# Autodesk Inventor assembly: 5-5
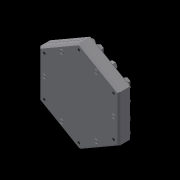
[picture p0: Inventor's stored thumbnail of the model, 180x180]
Saved by Autodesk Inventor 2017 (Build 210142000, 142)
## iProperties
Part Number: 5-5
Material: 一般
Document SubType Name: Assembly
Designer: r0909
Author: r0909
## Documents named in this file (7)
- C:\Users\r0909\Desktop\inventor\5-5.iam
- C:\Users\r0909\Desktop\inventor\5-1.ipt
- C:\Users\r0909\Desktop\inventor\5-2.ipt
- C:\Users\r0909\Desktop\inventor\5-3.ipt
- C:\Users\r0909\Desktop\inventor\5-4.ipt
- C:\Users\r0909\Desktop\inventor\5-5.1.ipt
- C:\Users\r0909\Desktop\inventor\5-5.2.ipt
## Components (44 placed, 6 different names)
1. 5-1:1 — 貼合:1, 貼合:2, 貼合:3, 貼合:30, 角度:19
2. 5-2:1 — 貼合:1, 貼合:2, 貼合:3, 貼合:4, 貼合:5, 貼合:6, 貼合:7, 貼合:8, 貼合:9, 齊平:1, 齊平:2, 齊平:3, 齊平:4, 齊平:5, 齊平:6, 貼合:12, 貼合:13, 角度:1, 貼合:24, 貼合:25, 貼合:26, 貼合:27, 貼合:28, 貼合:29, 角度:2, 貼合:31, 貼合:32, 貼合:33, 貼合:34, 貼合:35, 貼合:36, 貼合:37, 貼合:38, 貼合:39, 貼合:40, 貼合:41, 貼合:42, 貼合:43, 貼合:44, 貼合:45, 貼合:46, 貼合:47, 貼合:48, 貼合:49, 貼合:50, 貼合:51, 貼合:52, 貼合:53, 角度:6, 角度:11, 角度:12
3. 5-3:1 — 貼合:4, 齊平:1
4. 5-4:1 — 貼合:29, 貼合:30, 角度:2, 齊平:12, 齊平:13, 齊平:22, 角度:3
5. 5-3:2 — 貼合:5, 齊平:2
6. 5-3:3 — 貼合:6, 齊平:6
7. 5-3:4 — 貼合:7, 齊平:3
8. 5-3:5 — 貼合:8, 齊平:5
9. 5-3:6 — 貼合:9, 齊平:4
10. 5-5.1:1 — 貼合:10, 貼合:11, 貼合:13, 齊平:7
11. 5-5.2:1 — 貼合:10, 貼合:11, 貼合:12, 角度:1
12. 5-5.1:2 — 齊平:7, 齊平:8
13. 5-5.2:2 — 貼合:25
14. 5-5.1:3 — 齊平:8, 齊平:9
15. 5-5.2:3 — 貼合:24, 角度:7
16. 5-5.1:4 — 齊平:10, 齊平:11
17. 5-5.2:4 — 貼合:27
18. 5-5.1:5 — 齊平:9, 齊平:10
19. 5-5.2:5 — 貼合:26
20. 5-5.1:6 — 齊平:11
21. 5-5.2:6 — 貼合:28
22. 5-4:2 — 貼合:31, 齊平:22, 齊平:23, 角度:18
23. 5-4:3 — 貼合:34, 齊平:14, 角度:12, 角度:13
24. 5-4:4 — 貼合:33, 齊平:13, 齊平:14, 齊平:15, 齊平:16, 齊平:17, 角度:11
25. 5-4:5 — 貼合:32, 齊平:12, 角度:3, 角度:4
26. 5-4:6 — 貼合:35, 齊平:23, 齊平:24, 角度:17, 角度:18
27. 5-4:7 — 貼合:37, 齊平:24, 齊平:25, 角度:8, 角度:9
28. 5-4:8 — 貼合:36, 齊平:25, 齊平:26, 角度:6, 角度:7, 角度:8
29. 5-4:9 — 貼合:38, 齊平:16, 齊平:18
30. 5-4:10 — 貼合:39, 齊平:15
31. 5-4:11 — 貼合:48, 齊平:28, 齊平:29
32. 5-4:12 — 貼合:49, 齊平:32, 齊平:33, 角度:5
33. 5-4:13 — 貼合:47, 齊平:31, 角度:13, 角度:14, 角度:15
34. 5-4:14 — 貼合:46, 齊平:33, 齊平:34, 角度:4, 角度:5
35. 5-4:15 — 貼合:45, 齊平:34, 角度:16
36. 5-4:16 — 貼合:42, 齊平:20, 角度:10
37. 5-4:17 — 貼合:40, 齊平:17, 角度:22
38. 5-4:18 — 貼合:44, 齊平:21, 角度:15, 角度:16, 角度:17
39. 5-4:19 — 貼合:43, 齊平:19, 齊平:21, 角度:9, 角度:10
40. 5-4:20 — 貼合:41, 齊平:18, 齊平:19, 齊平:20, 角度:21, 角度:22
41. 5-4:21 — 貼合:53, 齊平:26, 齊平:27, 角度:20
42. 5-4:22 — 貼合:52, 齊平:27, 齊平:28, 角度:19, 角度:20, 角度:21
43. 5-4:23 — 貼合:51, 齊平:29, 齊平:30
44. 5-4:24 — 貼合:50, 齊平:30, 齊平:31, 齊平:32, 角度:14
## Relationships (109: Mate 53, Flush 34, Angle 22)
- 貼合:1 [Mate]: 5-1:1 ↔ 5-2:1
- 貼合:2 [Mate]: 5-1:1 ↔ 5-2:1
- 貼合:3 [Mate]: 5-1:1 ↔ 5-2:1
- 貼合:4 [Mate]: 5-2:1 ↔ 5-3:1
- 貼合:5 [Mate]: 5-2:1 ↔ 5-3:2
- 貼合:6 [Mate]: 5-2:1 ↔ 5-3:3
- 貼合:7 [Mate]: 5-2:1 ↔ 5-3:4
- 貼合:8 [Mate]: 5-2:1 ↔ 5-3:5
- 貼合:9 [Mate]: 5-2:1 ↔ 5-3:6
- 齊平:1 [Flush]: 5-2:1 ↔ 5-3:1
- 齊平:2 [Flush]: 5-2:1 ↔ 5-3:2
- 齊平:3 [Flush]: 5-2:1 ↔ 5-3:4
- 齊平:4 [Flush]: 5-2:1 ↔ 5-3:6
- 齊平:5 [Flush]: 5-2:1 ↔ 5-3:5
- 齊平:6 [Flush]: 5-2:1 ↔ 5-3:3
- 貼合:10 [Mate]: 5-5.1:1 ↔ 5-5.2:1
- 貼合:11 [Mate]: 5-5.1:1 ↔ 5-5.2:1
- 貼合:12 [Mate]: 5-2:1 ↔ 5-5.2:1
- 貼合:13 [Mate]: 5-2:1 ↔ 5-5.1:1
- 角度:1 [Angle] (0 deg): 5-2:1 ↔ 5-5.2:1
- [Mate]: 5-5.1:2 ↔ 5-5.2:2
- [Mate]: 5-5.1:2 ↔ 5-5.2:2
- [Mate]: 5-5.1:3 ↔ 5-5.2:3
- [Mate]: 5-5.1:3 ↔ 5-5.2:3
- [Mate]: 5-5.1:4 ↔ 5-5.2:4
- [Mate]: 5-5.1:4 ↔ 5-5.2:4
- [Mate]: 5-5.1:5 ↔ 5-5.2:5
- [Mate]: 5-5.1:5 ↔ 5-5.2:5
- [Mate]: 5-5.1:6 ↔ 5-5.2:6
- [Mate]: 5-5.1:6 ↔ 5-5.2:6
- 貼合:24 [Mate]: 5-2:1 ↔ 5-5.2:3
- 貼合:25 [Mate]: 5-2:1 ↔ 5-5.2:2
- 貼合:26 [Mate]: 5-2:1 ↔ 5-5.2:5
- 貼合:27 [Mate]: 5-2:1 ↔ 5-5.2:4
- 貼合:28 [Mate]: 5-2:1 ↔ 5-5.2:6
- 齊平:7 [Flush]: 5-5.1:1 ↔ 5-5.1:2
- 齊平:8 [Flush]: 5-5.1:2 ↔ 5-5.1:3
- 齊平:9 [Flush]: 5-5.1:3 ↔ 5-5.1:5
- 齊平:10 [Flush]: 5-5.1:4 ↔ 5-5.1:5
- 齊平:11 [Flush]: 5-5.1:4 ↔ 5-5.1:6
- 貼合:29 [Mate]: 5-2:1 ↔ 5-4:1
- 貼合:30 [Mate]: 5-1:1 ↔ 5-4:1
- 角度:2 [Angle] (0 deg): 5-2:1 ↔ 5-4:1
- 貼合:31 [Mate]: 5-2:1 ↔ 5-4:2
- 貼合:32 [Mate]: 5-2:1 ↔ 5-4:5
- 貼合:33 [Mate]: 5-2:1 ↔ 5-4:4
- 貼合:34 [Mate]: 5-2:1 ↔ 5-4:3
- 貼合:35 [Mate]: 5-2:1 ↔ 5-4:6
- 貼合:36 [Mate]: 5-2:1 ↔ 5-4:8
- 貼合:37 [Mate]: 5-2:1 ↔ 5-4:7
- 貼合:38 [Mate]: 5-2:1 ↔ 5-4:9
- 貼合:39 [Mate]: 5-2:1 ↔ 5-4:10
- 貼合:40 [Mate]: 5-2:1 ↔ 5-4:17
- 貼合:41 [Mate]: 5-2:1 ↔ 5-4:20
- 貼合:42 [Mate]: 5-2:1 ↔ 5-4:16
- 貼合:43 [Mate]: 5-2:1 ↔ 5-4:19
- 貼合:44 [Mate]: 5-2:1 ↔ 5-4:18
- 貼合:45 [Mate]: 5-2:1 ↔ 5-4:15
- 貼合:46 [Mate]: 5-2:1 ↔ 5-4:14
- 貼合:47 [Mate]: 5-2:1 ↔ 5-4:13
- 貼合:48 [Mate]: 5-2:1 ↔ 5-4:11
- 貼合:49 [Mate]: 5-2:1 ↔ 5-4:12
- 貼合:50 [Mate]: 5-2:1 ↔ 5-4:24
- 貼合:51 [Mate]: 5-2:1 ↔ 5-4:23
- 貼合:52 [Mate]: 5-2:1 ↔ 5-4:22
- 貼合:53 [Mate]: 5-2:1 ↔ 5-4:21
- 齊平:12 [Flush]: 5-4:1 ↔ 5-4:5
- 齊平:13 [Flush]: 5-4:1 ↔ 5-4:4
- 齊平:14 [Flush]: 5-4:3 ↔ 5-4:4
- 齊平:15 [Flush]: 5-4:4 ↔ 5-4:10
- 齊平:16 [Flush]: 5-4:4 ↔ 5-4:9
- 齊平:17 [Flush]: 5-4:4 ↔ 5-4:17
- 齊平:18 [Flush]: 5-4:9 ↔ 5-4:20
- 齊平:19 [Flush]: 5-4:19 ↔ 5-4:20
- 齊平:20 [Flush]: 5-4:16 ↔ 5-4:20
- 齊平:21 [Flush]: 5-4:18 ↔ 5-4:19
- 齊平:22 [Flush]: 5-4:1 ↔ 5-4:2
- 齊平:23 [Flush]: 5-4:2 ↔ 5-4:6
- 齊平:24 [Flush]: 5-4:6 ↔ 5-4:7
- 齊平:25 [Flush]: 5-4:7 ↔ 5-4:8
- 齊平:26 [Flush]: 5-4:8 ↔ 5-4:21
- 齊平:27 [Flush]: 5-4:21 ↔ 5-4:22
- 齊平:28 [Flush]: 5-4:11 ↔ 5-4:22
- 齊平:29 [Flush]: 5-4:11 ↔ 5-4:23
- 齊平:30 [Flush]: 5-4:23 ↔ 5-4:24
- 齊平:31 [Flush]: 5-4:13 ↔ 5-4:24
- 齊平:32 [Flush]: 5-4:12 ↔ 5-4:24
- 齊平:33 [Flush]: 5-4:12 ↔ 5-4:14
- 齊平:34 [Flush]: 5-4:14 ↔ 5-4:15
- 角度:3 [Angle] (0 deg): 5-4:1 ↔ 5-4:5
- 角度:4 [Angle] (0 deg): 5-4:5 ↔ 5-4:14
- 角度:5 [Angle] (0 deg): 5-4:12 ↔ 5-4:14
- 角度:6 [Angle] (0 deg): 5-2:1 ↔ 5-4:8
- 角度:7 [Angle] (0 deg): 5-5.2:3 ↔ 5-4:8
- 角度:8 [Angle] (0 deg): 5-4:7 ↔ 5-4:8
- 角度:9 [Angle] (0 deg): 5-4:7 ↔ 5-4:19
- 角度:10 [Angle] (0 deg): 5-4:16 ↔ 5-4:19
- 角度:11 [Angle] (0 deg): 5-2:1 ↔ 5-4:4
- 角度:12 [Angle] (0 deg): 5-2:1 ↔ 5-4:3
- 角度:13 [Angle] (0 deg): 5-4:3 ↔ 5-4:13
- 角度:14 [Angle] (0 deg): 5-4:13 ↔ 5-4:24
- 角度:15 [Angle] (0 deg): 5-4:13 ↔ 5-4:18
- 角度:16 [Angle] (0 deg): 5-4:15 ↔ 5-4:18
- 角度:17 [Angle] (0 deg): 5-4:6 ↔ 5-4:18
- 角度:18 [Angle] (0 deg): 5-4:2 ↔ 5-4:6
- 角度:19 [Angle] (0 deg): 5-1:1 ↔ 5-4:22
- 角度:20 [Angle] (0 deg): 5-4:21 ↔ 5-4:22
- 角度:21 [Angle] (0 deg): 5-4:20 ↔ 5-4:22
- 角度:22 [Angle] (0 deg): 5-4:17 ↔ 5-4:20
## Named parameters: d20_d16 = 0 mm, d21_d15 = 0 mm, d22_d16 = 0 mm, d23_d15 = 0 mm, d24_d16 = 0 mm, d25_d15 = 0 mm, d26_d16 = 0 mm, d27_d15 = 0 mm, d28_d16 = 0 mm, d29_d15 = 0 mm
